# Autodesk Inventor assembly: AssemblyCoxaKa
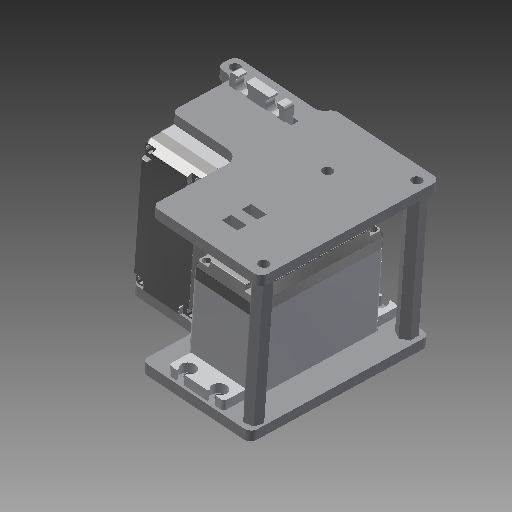
[picture p0: Inventor's stored thumbnail of the model, 512x512]
Saved by Autodesk Inventor 2019 (Build 230136000, 136)
## iProperties
Created: 2023-04-16
Part Number: AssemblyCoxaKa
Document SubType Name: Assembly
Designer: Analuam
Author: Analuam
## Documents named in this file (5)
- D:\Dek Diyah\AssemblyCoxaKa.iam
- D:\Dek Diyah\coxa.ipt
- D:\Dek Diyah\coxaa.ipt
- D:\Dek Diyah\Servo berputar.iam
- D:\Dek Diyah\spacer 5cm.ipt
## Components (7 placed, 4 different names)
1. Servo berputar:1 [sub-assembly] — Mate:1, Mate:2, Mate:3
2. coxa:1 — Mate:7, Mate:8, Mate:9, Insert:2, Insert:3
3. coxaa:1 — Mate:1, Mate:2, Mate:3, Mate:4, Mate:5, Mate:6, Insert:1
4. spacer 5cm:1 — Insert:1
5. Servo berputar:2 [sub-assembly] — Mate:4, Mate:5, Mate:6, Mate:7, Mate:8, Mate:9
6. spacer 5cm:2 — Insert:3
7. spacer 5cm:3 — Insert:2
## Relationships (12: Mate 9, Insert 3)
- Mate:1: Servo berputar:1 ↔ coxaa:1
- Mate:2: Servo berputar:1 ↔ coxaa:1
- Mate:3: Servo berputar:1 ↔ coxaa:1
- Mate:4: coxaa:1 ↔ Servo berputar:2
- Mate:5: coxaa:1 ↔ Servo berputar:2
- Mate:6: coxaa:1 ↔ Servo berputar:2
- Mate:7: coxa:1 ↔ Servo berputar:2
- Mate:8: coxa:1 ↔ Servo berputar:2
- Mate:9: coxa:1 ↔ Servo berputar:2
- Insert:1: coxaa:1 ↔ spacer 5cm:1
- Insert:2: coxa:1 ↔ spacer 5cm:3
- Insert:3: coxa:1 ↔ spacer 5cm:2
